# Autodesk Inventor assembly: E006-Carter
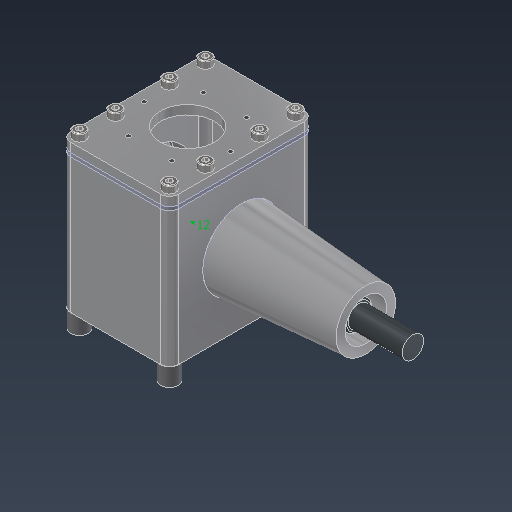
[picture p0: Inventor's stored thumbnail of the model, 512x512]
Saved by Autodesk Inventor 2021.3 (Build 253353000, 353)
## iProperties
Created: 2022-04-01
Part Number: E006-Carter
Document SubType Name: Assembly
Designer: remi
Author: remi
## Documents named in this file (19)
- C:\Users\remi\OneDrive\Documents\Cours\05-HEVS\S2fb\mechanic\CCo\project\Compressor\E006-Carter.iam
- C:\Users\remi\OneDrive\Documents\Cours\05-HEVS\S2fb\mechanic\CCo\project\Compressor\P016-Carter_corps.ipt
- C:\Users\remi\OneDrive\Documents\Cours\05-HEVS\S2fb\mechanic\CCo\project\Compressor\P015-Vilbrequin.ipt
- C:\Users\remi\OneDrive\Documents\Cours\05-HEVS\S2fb\mechanic\CCo\project\Compressor\P017-Carter_chapeau.ipt
- C:\Users\remi\OneDrive\Documents\Cours\05-HEVS\S2fb\mechanic\CCo\project\Compressor\P018-Joint_carter_chapeau.ipt
- C:\Users\remi\OneDrive\Documents\Cours\05-HEVS\S2fb\mechanic\CCo\project\Compressor\P020-Fixation_roulement_vilebrequin.ipt
- C:\Users\remi\OneDrive\Documents\Cours\05-HEVS\S2fb\mechanic\CCo\project\Compressor\R2021\en-US\AS 1420\AS 1420 - 1973 - M4 x 14.ipt
- C:\Users\remi\OneDrive\Documents\Cours\05-HEVS\S2fb\mechanic\CCo\project\Compressor\R2021\en-US\AS 1420\AS 1420 - 1973 - M4 x 8.ipt
- C:\Users\remi\OneDrive\Documents\Cours\05-HEVS\S2fb\mechanic\CCo\project\Compressor\P021-Bouchon_carter_vilbrequin.ipt
- C:\Users\remi\OneDrive\Documents\Cours\05-HEVS\S2fb\mechanic\CCo\project\Compressor\P022-Joint_carter_bouchon_vilbrequin.ipt
- C:\Users\remi\OneDrive\Documents\Cours\05-HEVS\S2fb\mechanic\CCo\project\Compressor\Roulements\AIS2021\SKF_W 61703-2RS1.iam
- C:\Users\remi\OneDrive\Documents\Cours\05-HEVS\S2fb\mechanic\CCo\project\Compressor\P024-Entretoise_roulements.ipt
- C:\Users\remi\OneDrive\Documents\Cours\05-HEVS\S2fb\mechanic\CCo\project\Compressor\E006-Carter\Design Accelerator\Key Connection2.iam
- C:\Users\remi\OneDrive\Documents\Cours\05-HEVS\S2fb\mechanic\CCo\project\Compressor\P025-Joint_carter_arbre.ipt
- C:\Users\remi\OneDrive\Documents\Cours\05-HEVS\S2fb\mechanic\CCo\project\Compressor\P026-Butée_carter_arbre.ipt
- C:\Users\remi\OneDrive\Documents\Cours\05-HEVS\S2fb\mechanic\CCo\project\Compressor\P023-Cage_arbre.ipt
- C:\Users\remi\OneDrive\Documents\Cours\05-HEVS\S2fb\mechanic\CCo\project\Compressor\R2021\en-US\AS 1420\AS 1420 - 1973 - M4 x 20.ipt
- C:\Users\remi\OneDrive\Documents\Cours\05-HEVS\S2fb\mechanic\CCo\project\Compressor\R2021\en-US\E 2076\_E 2076-10_.ipt
- C:\Users\remi\OneDrive\Documents\Cours\05-HEVS\S2fb\mechanic\CCo\project\Compressor\R2021\68978100.ipt
## Components (41 placed, 18 different names)
1. P016-Carter_corps:1 — Mate:6, Flush:1, Flush:2, Mate:9, Mate:10, Mate:11, Mate:16, Mate:22, Mate:23, Mate:24, Mate:25, Mate:28, Mate:31, Mate:35, Mate:37, Mate:38, Mate:39, Mate:40, Mate:41, Mate:42, Mate:43, Mate:44, Mate:45, Mate:46, Mate:47, Mate:48
2. P015-Vilbrequin:1 — Mate:7, Mate:8, Mate:14, Mate:15, Mate:18, Mate:20, Mate:31, Mate:34
3. P017-Carter_chapeau:1 — Mate:4, Mate:5, Flush:1, Flush:2, Insert:1, Insert:2, Insert:3, Insert:4, Insert:5, Insert:6, Insert:7, Insert:8
4. P018-Joint_carter_chapeau:1 — Mate:4, Mate:5, Mate:6
5. P020-Fixation_roulement_vilebrequin:1 — Mate:7, Mate:8, Insert:9
6. P021-Bouchon_carter_vilbrequin:1 — Mate:9, Mate:39, Mate:40, Insert:22, Insert:23, Insert:24, Insert:25, Insert:26, Insert:27
7. P022-Joint_carter_bouchon_vilbrequin:1 — Mate:10, Mate:11
8. P024-Entretoise_roulements:1 — Mate:20, Mate:21
9. Key Connection:1 [sub-assembly]
10. P025-Joint_carter_arbre:1 — Mate:22, Mate:25, Mate:32
11. P025-Joint_carter_arbre:2 — Mate:23, Mate:24, Mate:29, Mate:33
12. P026-Butée_carter_arbre:1 — Mate:28, Mate:29, Mate:30, Insert:16, Insert:17, Insert:18, Insert:19, Insert:20, Insert:21
13. P023-Cage_arbre:1 — Mate:34, Mate:35, Mate:36
14. AS 1420 - Metric M4 x 8:2 — Insert:22
15. AS 1420 - Metric M4 x 8:3 — Insert:23
16. AS 1420 - Metric M4 x 8:4 — Insert:24
17. AS 1420 - Metric M4 x 8:5 — Insert:25
18. AS 1420 - Metric M4 x 8:6 — Insert:26
19. AS 1420 - Metric M4 x 8:7 — Insert:27
20. AS 1420 - Metric M4 x 20:1 — Insert:16
21. AS 1420 - Metric M4 x 20:2 — Insert:17
22. AS 1420 - Metric M4 x 20:3 — Insert:18
23. AS 1420 - Metric M4 x 20:4 — Insert:19
24. AS 1420 - Metric M4 x 20:5 — Insert:20
25. AS 1420 - Metric M4 x 20:6 — Insert:21
26. AS 1420 - Metric M4 x 14:1 — Insert:1
27. AS 1420 - Metric M4 x 14:2 — Insert:2
28. AS 1420 - Metric M4 x 14:3 — Insert:3
29. AS 1420 - Metric M4 x 14:4 — Insert:4
30. AS 1420 - Metric M4 x 14:5 — Insert:5
31. AS 1420 - Metric M4 x 14:6 — Insert:6
32. AS 1420 - Metric M4 x 14:7 — Insert:7
33. AS 1420 - Metric M4 x 14:8 — Insert:8
34. AS 1420 - Metric M4 x 8:1 — Insert:9
35. SKF_W 61703-2RS1:1 [sub-assembly] — Mate:14, Mate:15, Mate:16, Mate:21
36. SKF_W 61703-2RS1:2 [sub-assembly] — Mate:18
37. E 2076 "14":1 — Mate:37, Mate:38
38. 68978100:1 — Mate:41, Mate:45
39. 68978100:2 — Mate:42, Mate:47
40. 68978100:3 — Mate:43, Mate:48
41. 68978100:4 — Mate:44, Mate:46
## Relationships (62: Mate 39, Insert 21, Flush 2)
- Mate:4: P017-Carter_chapeau:1 ↔ P018-Joint_carter_chapeau:1
- Mate:5: P017-Carter_chapeau:1 ↔ P018-Joint_carter_chapeau:1
- Mate:6: P016-Carter_corps:1 ↔ P018-Joint_carter_chapeau:1
- Flush:1: P016-Carter_corps:1 ↔ P017-Carter_chapeau:1
- Flush:2: P016-Carter_corps:1 ↔ P017-Carter_chapeau:1
- Mate:7: P015-Vilbrequin:1 ↔ P020-Fixation_roulement_vilebrequin:1
- Mate:8: P015-Vilbrequin:1 ↔ P020-Fixation_roulement_vilebrequin:1
- Insert:1: P017-Carter_chapeau:1 ↔ AS 1420 - Metric M4 x 14:1
- Insert:2: P017-Carter_chapeau:1 ↔ AS 1420 - Metric M4 x 14:2
- Insert:3: P017-Carter_chapeau:1 ↔ AS 1420 - Metric M4 x 14:3
- Insert:4: P017-Carter_chapeau:1 ↔ AS 1420 - Metric M4 x 14:4
- Insert:5: P017-Carter_chapeau:1 ↔ AS 1420 - Metric M4 x 14:5
- Insert:6: P017-Carter_chapeau:1 ↔ AS 1420 - Metric M4 x 14:6
- Insert:7: P017-Carter_chapeau:1 ↔ AS 1420 - Metric M4 x 14:7
- Insert:8: P017-Carter_chapeau:1 ↔ AS 1420 - Metric M4 x 14:8
- Insert:9: P020-Fixation_roulement_vilebrequin:1 ↔ AS 1420 - Metric M4 x 8:1
- Mate:9 (2 mm): P016-Carter_corps:1 ↔ P021-Bouchon_carter_vilbrequin:1
- Mate:10: P016-Carter_corps:1 ↔ P022-Joint_carter_bouchon_vilbrequin:1
- Mate:11: P016-Carter_corps:1 ↔ P022-Joint_carter_bouchon_vilbrequin:1
- Mate:14: P015-Vilbrequin:1 ↔ SKF_W 61703-2RS1:1
- Mate:15: P015-Vilbrequin:1 ↔ SKF_W 61703-2RS1:1
- Mate:16: P016-Carter_corps:1 ↔ SKF_W 61703-2RS1:1
- Mate:18: P015-Vilbrequin:1 ↔ SKF_W 61703-2RS1:2
- Mate:20: P015-Vilbrequin:1 ↔ P024-Entretoise_roulements:1
- Mate:21: P024-Entretoise_roulements:1 ↔ SKF_W 61703-2RS1:1
- Mate:22: P016-Carter_corps:1 ↔ P025-Joint_carter_arbre:1
- Mate:23: P016-Carter_corps:1 ↔ P025-Joint_carter_arbre:2
- Mate:24: P016-Carter_corps:1 ↔ P025-Joint_carter_arbre:2
- Mate:25: P016-Carter_corps:1 ↔ P025-Joint_carter_arbre:1
- Mate:28: P016-Carter_corps:1 ↔ P026-Butée_carter_arbre:1
- Mate:29: P025-Joint_carter_arbre:2 ↔ P026-Butée_carter_arbre:1
- Mate:30: P026-Butée_carter_arbre:1
- Mate:31: P016-Carter_corps:1 ↔ P015-Vilbrequin:1
- Mate:32: P025-Joint_carter_arbre:1
- Mate:33: P025-Joint_carter_arbre:2
- Mate:34: P015-Vilbrequin:1 ↔ P023-Cage_arbre:1
- Mate:35: P016-Carter_corps:1 ↔ P023-Cage_arbre:1
- Mate:36: P023-Cage_arbre:1
- Insert:16: P026-Butée_carter_arbre:1 ↔ AS 1420 - Metric M4 x 20:1
- Insert:17: P026-Butée_carter_arbre:1 ↔ AS 1420 - Metric M4 x 20:2
- Insert:18: P026-Butée_carter_arbre:1 ↔ AS 1420 - Metric M4 x 20:3
- Insert:19: P026-Butée_carter_arbre:1 ↔ AS 1420 - Metric M4 x 20:4
- Insert:20: P026-Butée_carter_arbre:1 ↔ AS 1420 - Metric M4 x 20:5
- Insert:21: P026-Butée_carter_arbre:1 ↔ AS 1420 - Metric M4 x 20:6
- Mate:37: P016-Carter_corps:1 ↔ E 2076 "14":1
- Mate:38: P016-Carter_corps:1 ↔ E 2076 "14":1
- Mate:39: P016-Carter_corps:1 ↔ P021-Bouchon_carter_vilbrequin:1
- Mate:40: P016-Carter_corps:1 ↔ P021-Bouchon_carter_vilbrequin:1
- Insert:22: P021-Bouchon_carter_vilbrequin:1 ↔ AS 1420 - Metric M4 x 8:2
- Insert:23: P021-Bouchon_carter_vilbrequin:1 ↔ AS 1420 - Metric M4 x 8:3
- Insert:24: P021-Bouchon_carter_vilbrequin:1 ↔ AS 1420 - Metric M4 x 8:4
- Insert:25: P021-Bouchon_carter_vilbrequin:1 ↔ AS 1420 - Metric M4 x 8:5
- Insert:26: P021-Bouchon_carter_vilbrequin:1 ↔ AS 1420 - Metric M4 x 8:6
- Insert:27: P021-Bouchon_carter_vilbrequin:1 ↔ AS 1420 - Metric M4 x 8:7
- Mate:41: P016-Carter_corps:1 ↔ 68978100:1
- Mate:42: P016-Carter_corps:1 ↔ 68978100:2
- Mate:43: P016-Carter_corps:1 ↔ 68978100:3
- Mate:44: P016-Carter_corps:1 ↔ 68978100:4
- Mate:45: P016-Carter_corps:1 ↔ 68978100:1
- Mate:46: P016-Carter_corps:1 ↔ 68978100:4
- Mate:47: P016-Carter_corps:1 ↔ 68978100:2
- Mate:48: P016-Carter_corps:1 ↔ 68978100:3
